# Autodesk Inventor assembly: batterybox
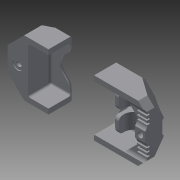
[picture p0: Inventor's stored thumbnail of the model, 180x180]
Saved by Autodesk Inventor 2014 (Build 180170000, 170)
## iProperties
Created: 2014-06-07
Part Number: batterybox
Document SubType Name: Assembly
Designer: brent
Author: brent
## Documents named in this file (3)
- C:\Users\brent\Documents\electric-longboard\brent\batterybox.iam
- C:\Users\brent\Documents\electric-longboard\brent\batterybox_front.ipt
- C:\Users\brent\Documents\electric-longboard\brent\batterybox_back.ipt
## Components (2 placed, 2 different names)
1. batterybox_front:1 — Flush:1, Mate:1, Flush:2
2. batterybox_back:1 — Flush:1, Mate:1, Flush:2
## Relationships (3: Flush 2, Mate 1)
- Flush:1: batterybox_front:1 ↔ batterybox_back:1
- Mate:1 (144.78 mm): batterybox_front:1 ↔ batterybox_back:1
- Flush:2: batterybox_front:1 ↔ batterybox_back:1
